# Autodesk Inventor assembly: Wheel
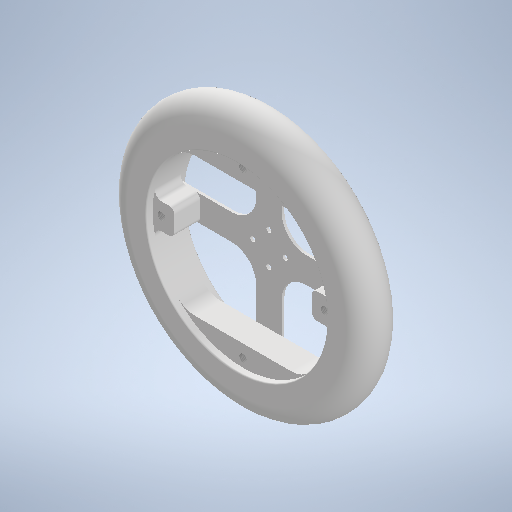
[picture p0: Inventor's stored thumbnail of the model, 512x512]
Saved by Autodesk Inventor 2025 (Build 290162000, 162)
## iProperties
Created: 2025-01-08
Part Number: Wheel
Document SubType Name: Assembly
Designer: 5014070
Author: 5014070
## Documents named in this file (3)
- C:\Users\5014070\Documents\GitHub\Mechanical\SeattleSolarCar2024-2025\Steering Wheel\Wheel.iam
- C:\Users\5014070\Documents\GitHub\Mechanical\SeattleSolarCar2024-2025\Steering Wheel\steering sheet.ipt
- C:\Users\5014070\Documents\GitHub\Mechanical\SeattleSolarCar2024-2025\Steering Wheel\steering wheel.ipt
## Components (2 placed, 2 different names)
1. steering sheet:1 — Mate:1, Mate:2, Mate:3
2. steering wheel:1 — Mate:1, Mate:2, Mate:3
## Relationships (3: Mate 3)
- Mate:1: steering sheet:1 ↔ steering wheel:1
- Mate:2: steering sheet:1 ↔ steering wheel:1
- Mate:3: steering sheet:1 ↔ steering wheel:1
